# Autodesk Inventor assembly: Overall_Assembly_Rev3
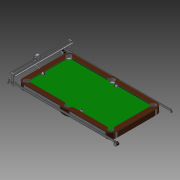
[picture p0: Inventor's stored thumbnail of the model, 180x180]
Saved by Autodesk Inventor 2015 (Build 190159000, 159)
## iProperties
Created: 2017-01-22
Part Number: Overall_Assembly_Rev3
Document SubType Name: Assembly
Designer: Guy
Author: Guy
## Documents named in this file (6)
- C:\Users\Guy\Documents\Fourth Year\Capstone\git\Capstone-Project\doc\CAD\LowLevel_Rev3\Overall_Assembly_Rev3.iam
- C:\Users\Guy\Documents\Fourth Year\Capstone\git\Capstone-Project\doc\CAD\Pool Table\Table_Model.ipt
- C:\Users\Guy\Documents\Fourth Year\Capstone\git\Capstone-Project\doc\CAD\LowLevel_Rev3\X_rail_Assembly_Rev3.iam
- C:\Users\Guy\Documents\Fourth Year\Capstone\git\Capstone-Project\doc\CAD\LowLevel_Rev3\Y_rail_Assembly_Rev3.iam
- C:\Users\Guy\Documents\Fourth Year\Capstone\git\Capstone-Project\doc\CAD\LowLevel_Rev3\Piston_Model.ipt
- C:\Users\Guy\Documents\Fourth Year\Capstone\git\Capstone-Project\doc\CAD\LowLevel_Rev2\Pool_Ball_Stripe.ipt
## Components (8 placed, 5 different names)
1. Table_Model:1 — Mate:2, Mate:4, Mate:5, Mate:7, Mate:8, Mate:9, Mate:15, Mate:16, Tangent:1, Tangent:2, Tangent:3, Tangent:4, Tangent:5, Tangent:6
2. X_rail_Assembly_Rev3:1 [sub-assembly] — Mate:2, Mate:4, Mate:5, Mate:7, Flush:1, Mate:16, Mate:17, Mate:18
3. X_rail_Assembly_Rev3:2 [sub-assembly] — Mate:8, Mate:9, Flush:1, Mate:15, Mate:19
4. Y_rail_Assembly_Rev3:1 [sub-assembly] — Mate:17, Mate:18, Mate:19, Mate:20, Flush:2
5. Piston_Model:1 — Mate:20, Flush:2
6. Pool_Ball_Stripe:1 — Tangent:1, Tangent:2
7. Pool_Ball_Stripe:2 — Tangent:3, Tangent:4
8. Pool_Ball_Stripe:3 — Tangent:5, Tangent:6
## Relationships (20: Mate 12, Tangent 6, Flush 2)
- Mate:2: Table_Model:1 ↔ X_rail_Assembly_Rev3:1
- Mate:4: Table_Model:1 ↔ X_rail_Assembly_Rev3:1
- Mate:5: Table_Model:1 ↔ X_rail_Assembly_Rev3:1
- Mate:7: Table_Model:1 ↔ X_rail_Assembly_Rev3:1
- Mate:8: Table_Model:1 ↔ X_rail_Assembly_Rev3:2
- Mate:9: Table_Model:1 ↔ X_rail_Assembly_Rev3:2
- Flush:1: X_rail_Assembly_Rev3:1 ↔ X_rail_Assembly_Rev3:2
- Mate:15 (50 mm): Table_Model:1 ↔ X_rail_Assembly_Rev3:2
- Mate:16 (50 mm): Table_Model:1 ↔ X_rail_Assembly_Rev3:1
- Mate:17: X_rail_Assembly_Rev3:1 ↔ Y_rail_Assembly_Rev3:1
- Mate:18: X_rail_Assembly_Rev3:1 ↔ Y_rail_Assembly_Rev3:1
- Mate:19: X_rail_Assembly_Rev3:2 ↔ Y_rail_Assembly_Rev3:1
- Mate:20: Y_rail_Assembly_Rev3:1 ↔ Piston_Model:1
- Tangent:1: Table_Model:1 ↔ Pool_Ball_Stripe:1
- Flush:2: Y_rail_Assembly_Rev3:1 ↔ Piston_Model:1
- Tangent:2: Table_Model:1 ↔ Pool_Ball_Stripe:1
- Tangent:3: Table_Model:1 ↔ Pool_Ball_Stripe:2
- Tangent:4: Table_Model:1 ↔ Pool_Ball_Stripe:2
- Tangent:5: Table_Model:1 ↔ Pool_Ball_Stripe:3
- Tangent:6: Table_Model:1 ↔ Pool_Ball_Stripe:3
